# Autodesk Inventor assembly: TransmissionLine
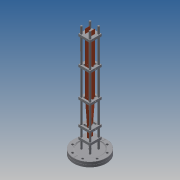
[picture p0: Inventor's stored thumbnail of the model, 180x180]
Saved by Autodesk Inventor 2015 (Build 190159000, 159)
## iProperties
Created: 2014-07-11
Part Number: TransmissionLine
Document SubType Name: Assembly
Designer: jad211
Author: jad211
## Documents named in this file (8)
- D:\Documents\Inventor\Microwave Transmission line\TransmissionLine.iam
- D:\Documents\Inventor\Microwave Transmission line\DN63CF blank cutout.ipt
- D:\Documents\Inventor\Microwave Transmission line\Rod.ipt
- D:\Documents\Inventor\Microwave Transmission line\Holder.ipt
- D:\Documents\Inventor\Microwave Transmission line\FieldPlates.ipt
- D:\Documents\Inventor\Microwave Transmission line\HolderStart.ipt
- D:\Documents\Inventor\Microwave Transmission line\HolderThin2.ipt
- D:\Documents\Inventor\Microwave Transmission line\HolderEnd.ipt
## Components (12 placed, 7 different names)
1. DN63CF blank cutout:1 — Mate:1, Mate:2, Mate:3, Mate:4, Mate:5, Mate:6, Mate:7, Mate:8, Mate:22, Mate:23, Flush:3, Flush:4
2. Rod:1 — Mate:7, Mate:8, Mate:30, Mate:32, Mate:39, Mate:44
3. Rod:2 — Mate:3, Mate:4, Mate:26, Mate:35, Mate:36, Mate:38, Mate:42
4. Rod:3 — Mate:5, Mate:6, Mate:27, Mate:31, Mate:34, Mate:37, Mate:41
5. Rod:4 — Mate:1, Mate:2, Mate:28, Mate:29, Mate:33, Mate:40, Mate:43
6. FieldPlates:1 — Flush:1, Mate:45, Flush:9
7. FieldPlates:2 — Mate:25, Mate:46, Flush:5, Flush:9
8. HolderStart:1 — Mate:26, Mate:27, Mate:28, Mate:45, Mate:46, Flush:5
9. HolderThin2:1 — Mate:29, Mate:30, Mate:31, Mate:36
10. Holder:1 — Mate:32, Mate:33, Mate:34, Mate:35, Flush:6
11. Holder:2 — Mate:41, Mate:42, Mate:43, Mate:44, Mate:47, Mate:48
12. HolderEnd:1 — Mate:37, Mate:38, Mate:39, Mate:40, Mate:48
## Relationships (41: Mate 34, Flush 7)
- Mate:1: DN63CF blank cutout:1 ↔ Rod:4
- Mate:2: DN63CF blank cutout:1 ↔ Rod:4
- Mate:3: DN63CF blank cutout:1 ↔ Rod:2
- Mate:4: DN63CF blank cutout:1 ↔ Rod:2
- Mate:5: DN63CF blank cutout:1 ↔ Rod:3
- Mate:6: DN63CF blank cutout:1 ↔ Rod:3
- Mate:7: DN63CF blank cutout:1 ↔ Rod:1
- Mate:8: DN63CF blank cutout:1 ↔ Rod:1
- Mate:22: DN63CF blank cutout:1
- Mate:23: DN63CF blank cutout:1
- Flush:1: FieldPlates:1
- Mate:25: FieldPlates:2
- Flush:3 (200 mm): DN63CF blank cutout:1
- Flush:4 (-15 mm): DN63CF blank cutout:1
- Mate:26: Rod:2 ↔ HolderStart:1
- Mate:27: Rod:3 ↔ HolderStart:1
- Mate:28: Rod:4 ↔ HolderStart:1
- Mate:29: Rod:4 ↔ HolderThin2:1
- Mate:30: Rod:1 ↔ HolderThin2:1
- Mate:31: Rod:3 ↔ HolderThin2:1
- Mate:32: Rod:1 ↔ Holder:1
- Mate:33: Rod:4 ↔ Holder:1
- Mate:34: Rod:3 ↔ Holder:1
- Mate:35: Rod:2 ↔ Holder:1
- Mate:36: Rod:2 ↔ HolderThin2:1
- Mate:37: Rod:3 ↔ HolderEnd:1
- Mate:38: Rod:2 ↔ HolderEnd:1
- Mate:39: Rod:1 ↔ HolderEnd:1
- Mate:40: Rod:4 ↔ HolderEnd:1
- Mate:41: Rod:3 ↔ Holder:2
- Mate:42: Rod:2 ↔ Holder:2
- Mate:43: Rod:4 ↔ Holder:2
- Mate:44: Rod:1 ↔ Holder:2
- Mate:45: FieldPlates:1 ↔ HolderStart:1
- Mate:46: FieldPlates:2 ↔ HolderStart:1
- Flush:5: FieldPlates:2 ↔ HolderStart:1
- Flush:6 (-45 mm): Holder:1
- Mate:47 (45 mm): Holder:2
- Flush:9: FieldPlates:1 ↔ FieldPlates:2
- Mate:48 (90 mm): Holder:2 ↔ HolderEnd:1
- Flush:10 (200 mm)
